# Autodesk Inventor assembly: sestava tělo estonsko s plechem otočené motory
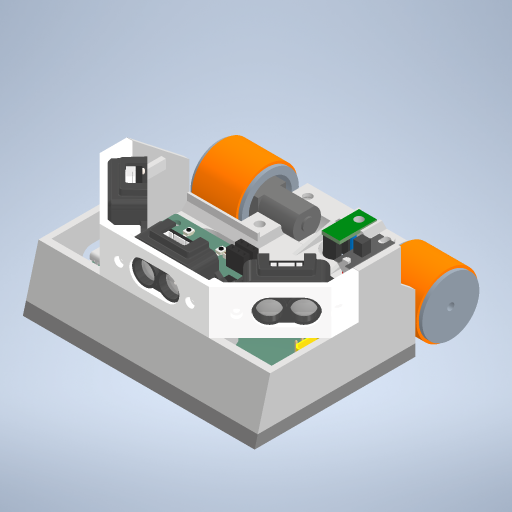
[picture p0: Inventor's stored thumbnail of the model, 512x512]
Saved by Autodesk Inventor 2024 (Build 280153000, 153)
## iProperties
Created: 2023-11-14
Part Number: sestava tělo estonsko s plechem otočené motory
Document SubType Name: Assembly
Designer: Simak
Author: Simak
## Documents named in this file (9)
- C:\Users\Simak\OneDrive\Dokumenty\GitHub\RoboCop\- 3D -\wip\Tělo s plechem\sestava tělo estonsko s plechem otočené motory.iam
- C:\Users\Simak\OneDrive\Dokumenty\GitHub\RoboCop\- 3D -\wip\Tělo s plechem\tělo estonsko s plechem otočené motory.ipt
- C:\Users\Simak\OneDrive\Dokumenty\GitHub\RoboCop\- 3D -\mech._parts\plech.ipt
- C:\Users\Simak\OneDrive\Dokumenty\GitHub\RoboCop\- 3D -\el._parts\sumec_smd.iam
- C:\Users\Simak\OneDrive\Dokumenty\GitHub\RoboCop\- 3D -\wip\Sestava TF-Luna a držáku.iam
- C:\Users\Simak\OneDrive\Dokumenty\GitHub\RoboCop\- 3D -\el._parts\qre_module.ipt
- C:\Users\Simak\OneDrive\Dokumenty\GitHub\RoboCop\- 3D -\el._parts\switch.ipt
- C:\Users\Simak\OneDrive\Dokumenty\GitHub\RoboCop\- 3D -\el._parts\GA12-N20_Motor.ipt
- C:\Users\Simak\OneDrive\Dokumenty\GitHub\RoboCop\- 3D -\mech._parts\wheel+silicon.ipt
## Components (10 placed, 8 different names)
1. tělo estonsko s plechem otočené motory:1 — Proti sobě:1, Stejný směr:1, Stejný směr:2, Proti sobě:2, Vložit:1, Vložit:2, Proti sobě:3, Proti sobě:4, Stejný směr:3, Vložit:3, Proti sobě:5, Proti sobě:6, Proti sobě:7, Proti sobě:8, Proti sobě:10, Proti sobě:11, Proti sobě:12, Proti sobě:13, Proti sobě:14, Proti sobě:15, Stejný směr:4, Stejný směr:5
2. plech:1 — Proti sobě:1, Stejný směr:1, Stejný směr:2
3. sumec_smd:1 [sub-assembly] — Proti sobě:2, Vložit:1, Vložit:2
4. Sestava TF-Luna a držáku:1 [sub-assembly] — Proti sobě:3, Proti sobě:4, Stejný směr:3
5. qre_module:1 — Vložit:3, Proti sobě:5
6. switch:1 — Proti sobě:6, Proti sobě:7, Proti sobě:8
7. GA12-N20_Motor:1 — Proti sobě:13, Proti sobě:14, Proti sobě:15, Proti sobě:17
8. GA12-N20_Motor:2 — Proti sobě:10, Proti sobě:11, Proti sobě:12, Proti sobě:16
9. wheel+silicon:1 — Stejný směr:5, Proti sobě:17
10. wheel+silicon:2 — Stejný směr:4, Proti sobě:16
## Relationships (24: Mate 16, Flush 5, Insert 3)
- Proti sobě:1 [Mate]: tělo estonsko s plechem otočené motory:1 ↔ plech:1
- Stejný směr:1 [Flush]: tělo estonsko s plechem otočené motory:1 ↔ plech:1
- Stejný směr:2 [Flush]: tělo estonsko s plechem otočené motory:1 ↔ plech:1
- Proti sobě:2 [Mate]: tělo estonsko s plechem otočené motory:1 ↔ sumec_smd:1
- Vložit:1 [Insert]: tělo estonsko s plechem otočené motory:1 ↔ sumec_smd:1
- Vložit:2 [Insert]: tělo estonsko s plechem otočené motory:1 ↔ sumec_smd:1
- Proti sobě:3 [Mate]: tělo estonsko s plechem otočené motory:1 ↔ Sestava TF-Luna a držáku:1
- Proti sobě:4 [Mate]: tělo estonsko s plechem otočené motory:1 ↔ Sestava TF-Luna a držáku:1
- Stejný směr:3 [Flush]: tělo estonsko s plechem otočené motory:1 ↔ Sestava TF-Luna a držáku:1
- Vložit:3 [Insert]: tělo estonsko s plechem otočené motory:1 ↔ qre_module:1
- Proti sobě:5 [Mate]: tělo estonsko s plechem otočené motory:1 ↔ qre_module:1
- Proti sobě:6 [Mate]: tělo estonsko s plechem otočené motory:1 ↔ switch:1
- Proti sobě:7 [Mate]: tělo estonsko s plechem otočené motory:1 ↔ switch:1
- Proti sobě:8 [Mate]: tělo estonsko s plechem otočené motory:1 ↔ switch:1
- Proti sobě:10 [Mate]: tělo estonsko s plechem otočené motory:1 ↔ GA12-N20_Motor:2
- Proti sobě:11 [Mate]: tělo estonsko s plechem otočené motory:1 ↔ GA12-N20_Motor:2
- Proti sobě:12 [Mate]: tělo estonsko s plechem otočené motory:1 ↔ GA12-N20_Motor:2
- Proti sobě:13 [Mate]: tělo estonsko s plechem otočené motory:1 ↔ GA12-N20_Motor:1
- Proti sobě:14 [Mate]: tělo estonsko s plechem otočené motory:1 ↔ GA12-N20_Motor:1
- Proti sobě:15 [Mate]: tělo estonsko s plechem otočené motory:1 ↔ GA12-N20_Motor:1
- Stejný směr:4 [Flush]: tělo estonsko s plechem otočené motory:1 ↔ wheel+silicon:2
- Proti sobě:16 [Mate]: GA12-N20_Motor:2 ↔ wheel+silicon:2
- Stejný směr:5 [Flush]: tělo estonsko s plechem otočené motory:1 ↔ wheel+silicon:1
- Proti sobě:17 [Mate]: GA12-N20_Motor:1 ↔ wheel+silicon:1
